# Autodesk Inventor assembly: Assembly2
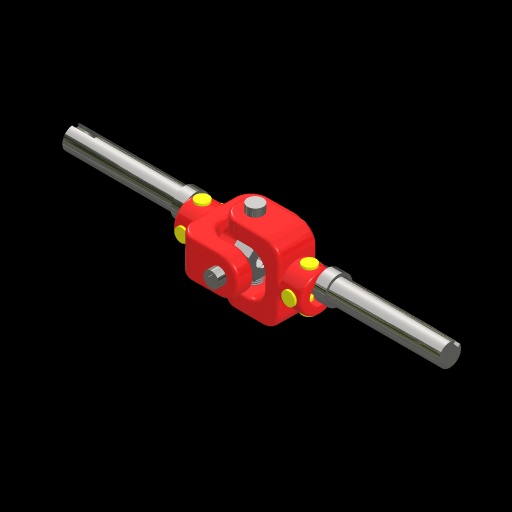
[picture p0: Inventor's stored thumbnail of the model, 512x512]
Saved by Autodesk Inventor 2024 (Build 280153000, 153)
## iProperties
Created: 2023-10-30
Part Number: Assembly2
Document SubType Name: Assembly
Designer: Admin
Author: Admin
## Documents named in this file (6)
- C:\Users\Administrator\Documents\AUTODESK\Exercise\class6.assembly\Assembly2.iam
- C:\Users\Administrator\Documents\AUTODESK\Exercise\class6.assembly\base.ipt
- C:\Users\Administrator\Documents\AUTODESK\Exercise\class6.assembly\bolt.ipt
- C:\Users\Administrator\Documents\AUTODESK\Exercise\class6.assembly\nut.ipt
- C:\Users\Administrator\Documents\AUTODESK\Exercise\class6.assembly\shaft.ipt
- C:\Users\Administrator\Documents\AUTODESK\Exercise\class6.assembly\pin.ipt
## Components (17 placed, 5 different names)
1. base:1 — Mate:6, Mate:10, Mate:11, Mate:15, Mate:16, Mate:20, Tangent:2, Mate:21, Rotation/Translation:1
2. bolt:1 — Mate:22, Tangent:4, Mate:26
3. bolt:2 — Mate:10, Mate:21
4. nut:1 — Mate:6, Mate:22, Mate:23, Mate:24, Rotation/Translation:1
5. base:2 — Mate:17, Mate:18, Mate:19, Tangent:1, Mate:24, Mate:25, Tangent:3, Tangent:4, Mate:26
6. bolt:3 — Mate:11, Flush:2
7. bolt:4 — Mate:23, Mate:25, Tangent:3
8. shaft:1 — Mate:17, Mate:18
9. shaft:2 — Mate:15, Mate:16
10. pin:8 — Mate:20, Tangent:2
11. pin:9
12. pin:10
13. pin:11
14. pin:7 — Mate:19, Tangent:1
15. pin:12
16. pin:13
17. pin:14
## Component patterns: (4 elements, first: pin:8), (4 elements, first: pin:7)
## Relationships (22: Mate 15, Tangent 4, Flush 2, RelateRotateTranslate 1)
- Mate:6: base:1 ↔ nut:1
- Mate:10: base:1 ↔ bolt:2
- Mate:11: base:1 ↔ bolt:3
- Mate:15: base:1 ↔ shaft:2
- Mate:16: base:1 ↔ shaft:2
- Mate:17: base:2 ↔ shaft:1
- Mate:18: base:2 ↔ shaft:1
- Mate:19: base:2 ↔ pin:7
- Tangent:1: base:2 ↔ pin:7
- Mate:20: base:1 ↔ pin:8
- Tangent:2: base:1 ↔ pin:8
- Mate:21: base:1 ↔ bolt:2
- Mate:22: bolt:1 ↔ nut:1
- Mate:23: nut:1 ↔ bolt:4
- Mate:24: nut:1 ↔ base:2
- Mate:25: base:2 ↔ bolt:4
- Tangent:3: base:2 ↔ bolt:4
- Tangent:4: bolt:1 ↔ base:2
- Mate:26: bolt:1 ↔ base:2
- Rotation/Translation:1 [RelateRotateTranslate] (59.69 mm): base:1 ↔ nut:1
- Flush:1 (-300 mm)
- Flush:2: bolt:3
